# Autodesk Inventor assembly: Frame 1647030135921
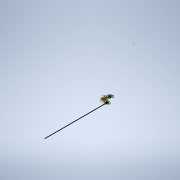
[picture p0: Inventor's stored thumbnail of the model, 180x180]
Saved by Autodesk Inventor 2022.2 (Build 262287010, 287A)
## iProperties
_FrameDoc: Frame Assembly
_Version: 25.0.0
Created: 2022-03-11
Part Number: Frame 1647030135921
Document SubType Name: Assembly
Designer: foriw
Mass: 6298.67 g
Surface Area: 9103.39 cm^2
Volume: 2238.81 cm^3
Density: 2.8134 g/cm^3
Author: foriw
## Documents named in this file (23)
- C:\Users\tobia\Documents\GitHub\BeerCart-CAD-Inventor\Workspaces\Workspace\beercart assembly - mekatronik\Frame\Frame 1647030135921.iam
- C:\Users\tobia\Documents\GitHub\BeerCart-CAD-Inventor\Workspaces\Workspace\beercart assembly - mekatronik\Frame\Skeleton 1647030135922.ipt
- C:\Users\tobia\Documents\GitHub\BeerCart-CAD-Inventor\Workspaces\Workspace\BackWheelMountingPlate.ipt
- C:\Users\tobia\Documents\GitHub\BeerCart-CAD-Inventor\Workspaces\Workspace\BackWheelMountingPlate_MIR_MIR.ipt
- C:\Users\tobia\Documents\GitHub\BeerCart-CAD-Inventor\Workspaces\Workspace\bearing housing front.ipt
- C:\Users\tobia\Documents\GitHub\BeerCart-CAD-Inventor\Workspaces\Workspace\beercart assembly - mekatronik\Frame\ISO 12633-2 20x20x2 1648573975084.ipt
- C:\Users\tobia\Documents\GitHub\BeerCart-CAD-Inventor\Workspaces\Workspace\BackWheelMountingPlate_MIR4.ipt
- C:\Users\tobia\Documents\GitHub\BeerCart-CAD-Inventor\Workspaces\Workspace\backWheelNoMotor brake mount.ipt
- C:\Users\tobia\Documents\GitHub\BeerCart-CAD-Inventor\Workspaces\Workspace\beercart assembly - mekatronik\Frame\ISO 12633-2 20x20x2 1649154464355.ipt
- C:\Users\tobia\Documents\GitHub\BeerCart-CAD-Inventor\Workspaces\Workspace\BackWheelMotorMountSpacer.ipt
- C:\Users\tobia\Documents\GitHub\BeerCart-CAD-Inventor\Workspaces\Workspace\beercart assembly - mekatronik\Frame\FrontWheelFrameNew.iam
- C:\Users\tobia\Documents\GitHub\BeerCart-CAD-Inventor\Workspaces\Workspace\headset bearing.ipt
- C:\Users\tobia\Documents\GitHub\BeerCart-CAD-Inventor\Workspaces\Workspace\bearing housing front_MIR.ipt
- C:\Users\tobia\Documents\GitHub\BeerCart-CAD-Inventor\Libraries\Content Center Files\en-US\ISO 7089\ISO 7089 - 6 - 140 HV(1).ipt
- C:\Users\tobia\Documents\GitHub\BeerCart-CAD-Inventor\Libraries\Content Center Files\en-US\ISO 4762(2)\ISO 4762 - M6 x 16ISO.ipt
- C:\Users\tobia\Documents\GitHub\BeerCart-CAD-Inventor\Workspaces\Workspace\rotating axel.ipt
- C:\Users\tobia\Documents\GitHub\BeerCart-CAD-Inventor\Workspaces\Workspace\beercart assembly - mekatronik\Frame\plan1 .iam
- C:\Users\tobia\Documents\GitHub\BeerCart-CAD-Inventor\Workspaces\Workspace\beercart assembly - mekatronik\Frame\Plan 2 øverste.iam
- C:\Users\tobia\Documents\GitHub\BeerCart-CAD-Inventor\Workspaces\Workspace\beercart assembly - mekatronik\Frame\plan 3 forgaffel stop'.iam
- C:\Users\tobia\Documents\GitHub\BeerCart-CAD-Inventor\Workspaces\Workspace\beercart assembly - mekatronik\Frame\plan 1 venstre side .iam
- C:\Users\tobia\Documents\GitHub\BeerCart-CAD-Inventor\Workspaces\Workspace\beercart assembly - mekatronik\Frame\Plan 4 venstre motor holder.iam
- C:\Users\tobia\Documents\GitHub\BeerCart-CAD-Inventor\Workspaces\Workspace\beercart assembly - mekatronik\Frame\plan 5 motor holder højre side.iam
- C:\Users\tobia\Documents\GitHub\BeerCart-CAD-Inventor\Workspaces\Workspace\beercart assembly - mekatronik\Frame\plan 6 front gaffel montage.iam
## Components (28 placed, 21 different names)
1. bearing housing front:1 — Mate:8, Insert:4, Mate:10, Mate:12
2. Reference Skeleton
3. BackWheelMountingPlate:1 — Flush:6, Rotational:2, Rigid:1
4. BackWheelMountingPlate_MIR_MIR:1
5. ISO 12633-2 20x20x2 - 105,43:1 — Flush:6, Rotational:2, Rigid:1
6. BackWheelMountingPlate_MIR4:1
7. backWheelNoMotor brake mount:1
8. ISO 12633-2 20x20x2 - 105,43:1
9. BackWheelMotorMountSpacer:1
10. FrontWheelFrameNew:1 [sub-assembly] — Insert:3, Mate:8, Insert:4, Angle:1
11. headset bearing:1 — Insert:3
12. bearing housing front_MIR:1 — Mate:14, Mate:16
13. ISO 7089 6:1 — Mate:10, Insert:5
14. ISO 4762 M6 x 16:1 — Insert:5
15. ISO 7089 6:2 — Mate:12, Insert:6
16. ISO 4762 M6 x 16:2 — Insert:6
17. ISO 7089 6:3 — Mate:14, Insert:7
18. ISO 4762 M6 x 16:3 — Insert:7
19. ISO 7089 6:4 — Mate:16, Insert:8
20. ISO 4762 M6 x 16:4 — Insert:8
21. rotating axel:1 — Flush:19, Angle:1
22. plan1 :1 [sub-assembly]
23. Plan 2 øverste:1 [sub-assembly]
24. plan 3 forgaffel stop':1 [sub-assembly]
25. plan 1 venstre side :1 [sub-assembly]
26. Plan 4 venstre motor holder:1 [sub-assembly]
27. plan 5 motor holder højre side:1 [sub-assembly]
28. plan 6 front gaffel montage:1 [sub-assembly]
## Relationships (17: Insert 6, Mate 6, Flush 2, RevoluteJoint 1, WeldJoint 1, Angle 1)
- Flush:6: BackWheelMountingPlate:1 ↔ ISO 12633-2 20x20x2 - 105,43:1
- Rotational:2 [RevoluteJoint]: BackWheelMountingPlate:1 ↔ ISO 12633-2 20x20x2 - 105,43:1
- Rigid:1 [WeldJoint]: BackWheelMountingPlate:1 ↔ ISO 12633-2 20x20x2 - 105,43:1
- Insert:3: FrontWheelFrameNew:1 ↔ headset bearing:1
- Mate:8: bearing housing front:1 ↔ FrontWheelFrameNew:1
- Insert:4: bearing housing front:1 ↔ FrontWheelFrameNew:1
- Mate:10: bearing housing front:1 ↔ ISO 7089 6:1
- Insert:5: ISO 7089 6:1 ↔ ISO 4762 M6 x 16:1
- Mate:12: bearing housing front:1 ↔ ISO 7089 6:2
- Insert:6: ISO 7089 6:2 ↔ ISO 4762 M6 x 16:2
- Mate:14: bearing housing front_MIR:1 ↔ ISO 7089 6:3
- Insert:7: ISO 7089 6:3 ↔ ISO 4762 M6 x 16:3
- Mate:16: bearing housing front_MIR:1 ↔ ISO 7089 6:4
- Insert:8: ISO 7089 6:4 ↔ ISO 4762 M6 x 16:4
- [Mate]: bearing housing front:1 ↔ rotating axel:1
- Flush:19: rotating axel:1
- Angle:1 (0 deg): FrontWheelFrameNew:1 ↔ rotating axel:1
## Named parameters: d99_d81 = 0 mm
